# Autodesk Inventor assembly: Сборка_куб
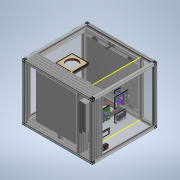
[picture p0: Inventor's stored thumbnail of the model, 180x180]
Saved by Autodesk Inventor 2020 (Build 240168000, 168)
## iProperties
Created: 2019-11-02
Part Number: Сборка_куб
Document SubType Name: Assembly
Designer: Михаил
Author: Михаил
## Documents named in this file (37)
- D:\MyWorks\GrowBox_v2\Box\3D_body\Сборка_куб.iam
- D:\MyWorks\GrowBox_v2\Box\3D_body\Профиль_аллюминиевый.ipt
- D:\MyWorks\GrowBox_v2\Box\3D_body\КубСоединительный2020.ipt
- D:\MyWorks\GrowBox_v2\Box\3D_body\Профиль_аллюминиевый460.ipt
- D:\MyWorks\GrowBox_v2\Box\3D_body\Профиль_аллюминиевый500.ipt
- D:\MyWorks\GrowBox_v2\Box\3D_body\Днище.ipt
- D:\MyWorks\GrowBox_v2\Box\3D_body\2004.ipt
- D:\MyWorks\GrowBox_v2\Box\3D_body\радиатор300х400.ipt
- D:\MyWorks\GrowBox_v2\Box\3D_body\ugolok40x40.ipt
- D:\MyWorks\GrowBox_v2\Box\3D_body\ugolok20x80.ipt
- D:\MyWorks\GrowBox_v2\Box\3D_body\petla.iam
- D:\MyWorks\GrowBox_v2\Box\3D_body\Uplotnitel-pazovyy400_-paz-6.ipt
- D:\MyWorks\GrowBox_v2\Box\3D_body\Uplotnitel-pazovyy380_-paz-6.ipt
- D:\MyWorks\GrowBox_v2\Box\3D_body\Uplotnitel-pazovyy500_-paz-6.ipt
- D:\MyWorks\GrowBox_v2\Box\3D_body\Дверка45.iam
- D:\MyWorks\GrowBox_v2\Box\3D_body\КрепежКулера.ipt
- D:\MyWorks\GrowBox_v2\Box\3D_body\NoctuaNF-A12x15.ipt
- D:\MyWorks\GrowBox_v2\Box\3D_body\КрепежРадиатора.ipt
- D:\MyWorks\GrowBox_v2\Box\3D_body\WaterContainer.ipt
- D:\MyWorks\GrowBox_v2\Box\3D_body\PowerSupply.ipt
- D:\MyWorks\GrowBox_v2\Box\3D_body\fitolamp_pcb.iam
- D:\MyWorks\GrowBox_v2\Box\3D_body\SensorsBoard.iam
- D:\MyWorks\GrowBox_v2\Box\3D_body\khadas-vim1-board.ipt
- D:\MyWorks\GrowBox_v2\Box\3D_body\Wall_Back_int.ipt
- D:\MyWorks\GrowBox_v2\Box\3D_body\DCDC_Holder.ipt
- D:\MyWorks\GrowBox_v2\Box\3D_body\FLC_Holder.ipt
- D:\MyWorks\GrowBox_v2\Box\3D_body\SensorsC_Holder.ipt
- D:\MyWorks\GrowBox_v2\Box\3D_body\SensorsBoard_3D\DA2_2.iam
- D:\MyWorks\GrowBox_v2\Box\3D_body\Wall_Input.ipt
- D:\MyWorks\GrowBox_v2\Box\3D_body\Wall_Output.ipt
- D:\MyWorks\GrowBox_v2\Box\3D_body\VIM1_Holder.ipt
- D:\MyWorks\GrowBox_v2\Box\3D_body\Wall_Front_door.ipt
- D:\MyWorks\GrowBox_v2\Box\3D_body\Разъем220.ipt
- D:\MyWorks\GrowBox_v2\Box\3D_body\Wall_Back_ext.ipt
- D:\MyWorks\GrowBox_v2\Box\3D_body\Wall_Top.ipt
- D:\MyWorks\GrowBox_v2\Box\3D_body\TempSensorHolder.ipt
- D:\MyWorks\GrowBox_v2\Box\3D_body\s-10-5_Holder.ipt
## Components (95 placed, 34 different names)
1. Профиль_алюминиевый:1 — Заподлицо:1, Заподлицо:2, Заподлицо:3, Совмещение:1, Заподлицо:4, Заподлицо:5, Совмещение:2, Заподлицо:6, Заподлицо:7
2. КубСоединительный2020:1 — Совмещение:1, Заподлицо:4, Заподлицо:5, Совмещение:6, Заподлицо:15, Совмещение:8, Заподлицо:18, Заподлицо:19, Заподлицо:20
3. КубСоединительный2020:2 — Совмещение:10, Заподлицо:23, Заподлицо:24, Совмещение:28, Заподлицо:50, Совмещение:29, Заподлицо:52, Заподлицо:53
4. КубСоединительный2020:3 — Совмещение:11, Заподлицо:25, Заподлицо:26, Заподлицо:51, Совмещение:30, Заподлицо:54, Заподлицо:55
5. КубСоединительный2020:4 — Совмещение:2, Заподлицо:6, Заподлицо:7, Совмещение:7, Заподлицо:16, Заподлицо:17, Совмещение:9, Заподлицо:21, Заподлицо:22
6. Профиль_алюминиевый:5 — Совмещение:7, Заподлицо:16, Заподлицо:17, Совмещение:13, Совмещение:15, Совмещение:16, Совмещение:34, Заподлицо:62, Заподлицо:63, Совмещение:53, Совмещение:91, Совмещение:104
7. Профиль_алюминиевый:6 — Совмещение:6, Заподлицо:15, Совмещение:31, Заподлицо:56, Заподлицо:57, Совмещение:56, Совмещение:71, Заподлицо:96, Совмещение:72, Заподлицо:97, Совмещение:85, Совмещение:96, Совмещение:105
8. Профиль_алюминиевый:7 — Совмещение:8, Заподлицо:18, Заподлицо:19, Заподлицо:20, Совмещение:10, Заподлицо:23, Заподлицо:24, Совмещение:20, Заподлицо:34, Заподлицо:35
9. Профиль_алюминиевый:8 — Совмещение:9, Заподлицо:21, Заподлицо:22, Совмещение:11, Заподлицо:25, Заподлицо:26, Совмещение:12, Заподлицо:27, Заподлицо:115
10. Профиль_алюминиевый:9 — Совмещение:12, Совмещение:13, Заподлицо:27, Совмещение:14, Заподлицо:28
11. Профиль_алюминиевый:10 — Совмещение:14, Совмещение:15, Заподлицо:28, Заподлицо:29, Совмещение:17, Совмещение:24, Заподлицо:43
12. Профиль_алюминиевый:11 — Совмещение:16, Заподлицо:29, Совмещение:17, Заподлицо:42, Заподлицо:86, Совмещение:54
13. Профиль_алюминиевый:12 — Заподлицо:32, Совмещение:20, Заподлицо:34, Заподлицо:35, Совмещение:114
14. Профиль_алюминиевый:13 — Заподлицо:32, Заподлицо:33
15. Профиль_алюминиевый:14 — Заподлицо:33, Совмещение:55, Заподлицо:87
16. Профиль_алюминиевый:15 — Заподлицо:36, Заподлицо:41, Совмещение:21, Совмещение:115, Заподлицо:116
17. Профиль_алюминиевый:16 — Заподлицо:36, Заподлицо:37, Заподлицо:40, Заподлицо:41, Совмещение:21, Совмещение:22, Совмещение:118
18. Профиль_алюминиевый:17 — Заподлицо:37, Заподлицо:38, Заподлицо:39, Заподлицо:40, Совмещение:22, Совмещение:23, Заподлицо:43
19. Профиль_алюминиевый:18 — Заподлицо:38, Заподлицо:39, Совмещение:23, Совмещение:24, Заподлицо:42, Совмещение:57, Заподлицо:88
20. Профиль_алюминиевый:19 — Заподлицо:50, Заподлицо:51
21. Профиль_алюминиевый:20 — Совмещение:28
22. Профиль_алюминиевый:21
23. Профиль_алюминиевый:22 — Совмещение:76, Заподлицо:99, Совмещение:144, Заподлицо:132
24. Профиль_алюминиевый:23 — Совмещение:30, Заподлицо:54, Заподлицо:55, Совмещение:33, Заподлицо:60, Заподлицо:61, Совмещение:79, Совмещение:89
25. Профиль_алюминиевый:24 — Совмещение:29, Заподлицо:52, Заподлицо:53, Совмещение:32, Заподлицо:58, Заподлицо:59, Совмещение:81, Совмещение:87
26. КубСоединительный2020:5 — Совмещение:34, Заподлицо:62, Заподлицо:63, Совмещение:35, Заподлицо:64, Заподлицо:65, Совмещение:92
27. КубСоединительный2020:6 — Совмещение:33, Заподлицо:60, Заподлицо:61, Совмещение:38, Заподлицо:70, Заподлицо:71, Совмещение:80, Совмещение:90, Совмещение:131
28. КубСоединительный2020:7 — Совмещение:32, Заподлицо:58, Заподлицо:59, Совмещение:37, Заподлицо:68, Заподлицо:69, Заподлицо:76, Совмещение:78, Совмещение:82, Совмещение:88
29. КубСоединительный2020:8 — Совмещение:31, Заподлицо:56, Заподлицо:57, Совмещение:36, Заподлицо:66, Заподлицо:67, Совмещение:86, Совмещение:129
30. Профиль_алюминиевый:25 — Совмещение:35, Заподлицо:64, Заподлицо:65, Совмещение:49, Заподлицо:84, Совмещение:97, Совмещение:109, Заподлицо:131
31. Профиль_алюминиевый:26 — Совмещение:36, Заподлицо:66, Заподлицо:67, Совмещение:44, Заподлицо:75, Заподлицо:76, Совмещение:45, Заподлицо:77, Совмещение:52, Совмещение:128, Заподлицо:130
32. Профиль_алюминиевый:27 — Совмещение:38, Заподлицо:70, Заподлицо:71, Совмещение:43, Заподлицо:74, Совмещение:50, Совмещение:103, Совмещение:117, Совмещение:130, Совмещение:143
33. Профиль_алюминиевый:28 — Совмещение:37, Заподлицо:68, Заподлицо:69, Совмещение:46, Совмещение:77, Заподлицо:129
34. Днище:1 — Совмещение:98, Совмещение:99, Совмещение:100
35. Профиль_алюминиевый:29 — Совмещение:45, Заподлицо:77, Совмещение:46, Заподлицо:78, Заподлицо:79, Совмещение:51, Заподлицо:85, Совмещение:84, Заподлицо:101
36. 2004:1 — Совмещение:43, Заподлицо:74, Заподлицо:79
37. 2004:2 — Совмещение:44, Заподлицо:75, Заподлицо:78
38. Профиль_алюминиевый:30 — Совмещение:47, Заподлицо:80, Заподлицо:81, Совмещение:49, Заподлицо:84, Совмещение:50
39. Профиль_алюминиевый:31 — Совмещение:47, Заподлицо:80, Заподлицо:81, Совмещение:108, Заподлицо:110
40. Профиль_алюминиевый:32 — Заподлицо:85, Совмещение:52, Совмещение:145, Заподлицо:133
41. Профиль_алюминиевый:33 — Совмещение:51
42. радиатор300х400:1 — Совмещение:108, Заподлицо:110, Совмещение:109, Совмещение:110, Заподлицо:111, Совмещение:111, Заподлицо:112, Совмещение:112, Заподлицо:113, Совмещение:113, Заподлицо:114
43. Профиль_алюминиевый:34 — Заподлицо:86, Совмещение:53, Совмещение:54, Совмещение:63, Заподлицо:89, Заподлицо:90, Совмещение:67, Совмещение:94, Заподлицо:103, Заподлицо:104, Заподлицо:127
44. Профиль_алюминиевый:35 — Совмещение:55, Заподлицо:87, Совмещение:56, Совмещение:58, Совмещение:64, Заподлицо:91, Совмещение:66, Заподлицо:92, Совмещение:93, Заподлицо:102, Совмещение:99, Совмещение:102, Заподлицо:105, Совмещение:116, Заподлицо:126
45. Профиль_алюминиевый:36 — Совмещение:57, Совмещение:58, Заподлицо:88, Совмещение:65, Совмещение:68, Заподлицо:93, Совмещение:69, Заподлицо:94, Совмещение:70, Заподлицо:95, Совмещение:83, Заподлицо:100, Совмещение:100, Заподлицо:125
46. ugolok40x40:1 — Совмещение:63, Заподлицо:89, Заподлицо:90
47. ugolok40x40:2 — Совмещение:67, Совмещение:68, Заподлицо:93
48. ugolok40x40:3 — Совмещение:65, Совмещение:66, Заподлицо:92
49. ugolok40x40:4 — Совмещение:64, Заподлицо:91, Совмещение:98
50. ugolok20x80:1 — Совмещение:69, Заподлицо:94
51. ugolok20x80:2 — Совмещение:70, Заподлицо:95
52. petla:1 [sub-assembly] — Совмещение:71, Заподлицо:96, Совмещение:95
53. petla:2 [sub-assembly] — Совмещение:72, Заподлицо:97
54. Uplotnitel-pazovyy400_-paz-6:1 — Совмещение:76, Заподлицо:99
55. Uplotnitel-pazovyy400_-paz-6:2 — Совмещение:77, Совмещение:78, Совмещение:142
56. Uplotnitel-pazovyy400_-paz-6:3 — Совмещение:79, Совмещение:80, Совмещение:141
57. Uplotnitel-pazovyy400_-paz-6:4 — Совмещение:81, Совмещение:82
58. Uplotnitel-pazovyy400_-paz-6:5 — Совмещение:83, Заподлицо:100
59. Uplotnitel-pazovyy400_-paz-6:6 — Совмещение:84, Заподлицо:101
60. Uplotnitel-pazovyy380_-paz-6:1 — Совмещение:87, Совмещение:88
61. Uplotnitel-pazovyy380_-paz-6:2 — Совмещение:85, Совмещение:86, Совмещение:133
62. Uplotnitel-pazovyy380_-paz-6:3 — Совмещение:89, Совмещение:90
63. Uplotnitel-pazovyy380_-paz-6:4 — Совмещение:91, Совмещение:92, Совмещение:135
64. Uplotnitel-pazovyy500_-paz-6:1 — Совмещение:93, Заподлицо:102, Совмещение:132
65. Uplotnitel-pazovyy500_-paz-6:2 — Совмещение:94, Заподлицо:103
66. Дверка45:1 [sub-assembly] — Совмещение:95, Совмещение:96, Совмещение:97, Совмещение:138, Совмещение:139, Заподлицо:128
67. КрепежКулера:1 — Совмещение:102, Заподлицо:105, Совмещение:105, Совмещение:107, Заподлицо:108, Заподлицо:109
68. КрепежКулера:2 — Заподлицо:104, Совмещение:103, Совмещение:104, Совмещение:106, Заподлицо:106, Заподлицо:107
69. NoctuaNF-A12x15:1 — Совмещение:106, Заподлицо:106, Заподлицо:107
70. NoctuaNF-A12x15:2 — Совмещение:107, Заподлицо:108, Заподлицо:109
71. КрепежРадиатора:1 — Совмещение:111, Заподлицо:112
72. КрепежРадиатора:2 — Совмещение:110, Заподлицо:111
73. КрепежРадиатора:3 — Совмещение:112, Заподлицо:113
74. КрепежРадиатора:4 — Совмещение:113, Заподлицо:114
75. WaterContainer:1 — Совмещение:114, Совмещение:115, Заподлицо:115
76. PowerSupply:1 — Совмещение:118, Заподлицо:116
77. fitolamp_pcb:1 [sub-assembly] — Совмещение:124, Заподлицо:117, Заподлицо:118
78. SensorsBoard:1 [sub-assembly] — Совмещение:126, Заподлицо:119, Заподлицо:120
79. khadas-vim1-board:1 — Совмещение:136, Заподлицо:123, Заподлицо:124
80. Wall_Back_int:1 — Совмещение:116, Совмещение:117, Совмещение:122, Совмещение:123, Совмещение:125, Совмещение:137, Совмещение:140, Заподлицо:125, Совмещение:146
81. DCDC_Holder:1 — Совмещение:122, Совмещение:127, Заподлицо:121, Заподлицо:122
82. FLC_Holder:1 — Совмещение:123, Совмещение:124, Заподлицо:117, Заподлицо:118
83. SensorsC_Holder:1 — Совмещение:125, Совмещение:126, Заподлицо:119, Заподлицо:120
84. DA2_2:1 [sub-assembly] — Совмещение:127, Заподлицо:121, Заподлицо:122
85. Uplotnitel-pazovyy500_-paz-6:3 — Совмещение:128, Совмещение:129
86. Uplotnitel-pazovyy500_-paz-6:4 — Совмещение:130, Совмещение:131, Совмещение:134
87. Wall_Input:1 — Совмещение:132, Совмещение:133, Совмещение:140, Заподлицо:126
88. Wall_Output:1 — Совмещение:134, Совмещение:135, Заподлицо:127
89. VIM1_Holder:1 — Совмещение:136, Заподлицо:123, Заподлицо:124, Совмещение:137
90. Wall_Front_door:1 — Совмещение:138, Совмещение:139, Заподлицо:128
91. Разъем220:1 — Совмещение:144, Заподлицо:132
92. Wall_Back_ext:1 — Заподлицо:129, Совмещение:141, Совмещение:142
93. Wall_Top:1 — Заподлицо:130, Совмещение:143, Заподлицо:131
94. TempSensorHolder:1 — Совмещение:145, Заподлицо:133
95. s-10-5_Holder:1 — Совмещение:146
## Relationships (251: Mate 128, Flush 123)
- Заподлицо:1 [Flush] (-6.75 mm): Профиль_алюминиевый:1
- Заподлицо:2 [Flush] (206.363 mm): Профиль_алюминиевый:1
- Заподлицо:3 [Flush] (17.615 mm): Профиль_алюминиевый:1
- Совмещение:1 [Mate]: Профиль_алюминиевый:1 ↔ КубСоединительный2020:1
- Заподлицо:4 [Flush]: Профиль_алюминиевый:1 ↔ КубСоединительный2020:1
- Заподлицо:5 [Flush]: Профиль_алюминиевый:1 ↔ КубСоединительный2020:1
- Совмещение:2 [Mate]: Профиль_алюминиевый:1 ↔ КубСоединительный2020:4
- Заподлицо:6 [Flush]: Профиль_алюминиевый:1 ↔ КубСоединительный2020:4
- Заподлицо:7 [Flush]: Профиль_алюминиевый:1 ↔ КубСоединительный2020:4
- Совмещение:6 [Mate]: КубСоединительный2020:1 ↔ Профиль_алюминиевый:6
- Заподлицо:15 [Flush]: КубСоединительный2020:1 ↔ Профиль_алюминиевый:6
- Совмещение:7 [Mate]: КубСоединительный2020:4 ↔ Профиль_алюминиевый:5
- Заподлицо:16 [Flush]: КубСоединительный2020:4 ↔ Профиль_алюминиевый:5
- Заподлицо:17 [Flush]: КубСоединительный2020:4 ↔ Профиль_алюминиевый:5
- Совмещение:8 [Mate]: КубСоединительный2020:1 ↔ Профиль_алюминиевый:7
- Заподлицо:18 [Flush]: КубСоединительный2020:1 ↔ Профиль_алюминиевый:7
- Заподлицо:19 [Flush]: КубСоединительный2020:1 ↔ Профиль_алюминиевый:7
- Заподлицо:20 [Flush]: КубСоединительный2020:1 ↔ Профиль_алюминиевый:7
- Совмещение:9 [Mate]: КубСоединительный2020:4 ↔ Профиль_алюминиевый:8
- Заподлицо:21 [Flush]: КубСоединительный2020:4 ↔ Профиль_алюминиевый:8
- Заподлицо:22 [Flush]: КубСоединительный2020:4 ↔ Профиль_алюминиевый:8
- Совмещение:10 [Mate]: КубСоединительный2020:2 ↔ Профиль_алюминиевый:7
- Заподлицо:23 [Flush]: КубСоединительный2020:2 ↔ Профиль_алюминиевый:7
- Заподлицо:24 [Flush]: КубСоединительный2020:2 ↔ Профиль_алюминиевый:7
- Совмещение:11 [Mate]: КубСоединительный2020:3 ↔ Профиль_алюминиевый:8
- Заподлицо:25 [Flush]: КубСоединительный2020:3 ↔ Профиль_алюминиевый:8
- Заподлицо:26 [Flush]: КубСоединительный2020:3 ↔ Профиль_алюминиевый:8
- Совмещение:12 [Mate]: Профиль_алюминиевый:8 ↔ Профиль_алюминиевый:9
- Совмещение:13 [Mate]: Профиль_алюминиевый:5 ↔ Профиль_алюминиевый:9
- Заподлицо:27 [Flush]: Профиль_алюминиевый:8 ↔ Профиль_алюминиевый:9
- Совмещение:14 [Mate]: Профиль_алюминиевый:9 ↔ Профиль_алюминиевый:10
- Совмещение:15 [Mate]: Профиль_алюминиевый:5 ↔ Профиль_алюминиевый:10
- Заподлицо:28 [Flush]: Профиль_алюминиевый:9 ↔ Профиль_алюминиевый:10
- Совмещение:16 [Mate]: Профиль_алюминиевый:5 ↔ Профиль_алюминиевый:11
- Заподлицо:29 [Flush]: Профиль_алюминиевый:10 ↔ Профиль_алюминиевый:11
- Совмещение:17 [Mate]: Профиль_алюминиевый:10 ↔ Профиль_алюминиевый:11
- [Mate]: Профиль_алюминиевый:12 ↔ Профиль_алюминиевый:13
- [Flush]: Профиль_алюминиевый:12 ↔ Профиль_алюминиевый:13
- [Flush]: Профиль_алюминиевый:13 ↔ Профиль_алюминиевый:14
- [Mate]: Профиль_алюминиевый:13 ↔ Профиль_алюминиевый:14
- Заподлицо:32 [Flush]: Профиль_алюминиевый:12 ↔ Профиль_алюминиевый:13
- Заподлицо:33 [Flush]: Профиль_алюминиевый:13 ↔ Профиль_алюминиевый:14
- Совмещение:20 [Mate]: Профиль_алюминиевый:7 ↔ Профиль_алюминиевый:12
- Заподлицо:34 [Flush]: Профиль_алюминиевый:7 ↔ Профиль_алюминиевый:12
- Заподлицо:35 [Flush]: Профиль_алюминиевый:7 ↔ Профиль_алюминиевый:12
- Заподлицо:36 [Flush]: Профиль_алюминиевый:15 ↔ Профиль_алюминиевый:16
- Заподлицо:37 [Flush]: Профиль_алюминиевый:16 ↔ Профиль_алюминиевый:17
- Заподлицо:38 [Flush]: Профиль_алюминиевый:17 ↔ Профиль_алюминиевый:18
- Заподлицо:39 [Flush]: Профиль_алюминиевый:17 ↔ Профиль_алюминиевый:18
- Заподлицо:40 [Flush]: Профиль_алюминиевый:16 ↔ Профиль_алюминиевый:17
- Заподлицо:41 [Flush]: Профиль_алюминиевый:15 ↔ Профиль_алюминиевый:16
- Совмещение:21 [Mate]: Профиль_алюминиевый:15 ↔ Профиль_алюминиевый:16
- Совмещение:22 [Mate]: Профиль_алюминиевый:16 ↔ Профиль_алюминиевый:17
- Совмещение:23 [Mate]: Профиль_алюминиевый:17 ↔ Профиль_алюминиевый:18
- Совмещение:24 [Mate]: Профиль_алюминиевый:10 ↔ Профиль_алюминиевый:18
- Заподлицо:42 [Flush]: Профиль_алюминиевый:11 ↔ Профиль_алюминиевый:18
- Заподлицо:43 [Flush] (80 mm): Профиль_алюминиевый:10 ↔ Профиль_алюминиевый:17
- [Flush]: Профиль_алюминиевый:19 ↔ Профиль_алюминиевый:20
- [Flush]: Профиль_алюминиевый:20 ↔ Профиль_алюминиевый:21
- [Flush]: Профиль_алюминиевый:21 ↔ Профиль_алюминиевый:22
- [Flush]: Профиль_алюминиевый:21 ↔ Профиль_алюминиевый:22
- [Flush]: Профиль_алюминиевый:20 ↔ Профиль_алюминиевый:21
- [Flush]: Профиль_алюминиевый:19 ↔ Профиль_алюминиевый:20
- [Mate]: Профиль_алюминиевый:19 ↔ Профиль_алюминиевый:20
- [Mate]: Профиль_алюминиевый:20 ↔ Профиль_алюминиевый:21
- [Mate]: Профиль_алюминиевый:21 ↔ Профиль_алюминиевый:22
- Совмещение:28 [Mate]: КубСоединительный2020:2 ↔ Профиль_алюминиевый:20
- Заподлицо:50 [Flush]: КубСоединительный2020:2 ↔ Профиль_алюминиевый:19
- Заподлицо:51 [Flush]: КубСоединительный2020:3 ↔ Профиль_алюминиевый:19
- Совмещение:29 [Mate]: КубСоединительный2020:2 ↔ Профиль_алюминиевый:24
- Заподлицо:52 [Flush]: КубСоединительный2020:2 ↔ Профиль_алюминиевый:24
- Заподлицо:53 [Flush]: КубСоединительный2020:2 ↔ Профиль_алюминиевый:24
- Совмещение:30 [Mate]: КубСоединительный2020:3 ↔ Профиль_алюминиевый:23
- Заподлицо:54 [Flush]: КубСоединительный2020:3 ↔ Профиль_алюминиевый:23
- Заподлицо:55 [Flush]: КубСоединительный2020:3 ↔ Профиль_алюминиевый:23
- Совмещение:31 [Mate]: Профиль_алюминиевый:6 ↔ КубСоединительный2020:8
- Заподлицо:56 [Flush]: Профиль_алюминиевый:6 ↔ КубСоединительный2020:8
- Заподлицо:57 [Flush]: Профиль_алюминиевый:6 ↔ КубСоединительный2020:8
- Совмещение:32 [Mate]: Профиль_алюминиевый:24 ↔ КубСоединительный2020:7
- Заподлицо:58 [Flush]: Профиль_алюминиевый:24 ↔ КубСоединительный2020:7
- Заподлицо:59 [Flush]: Профиль_алюминиевый:24 ↔ КубСоединительный2020:7
- Совмещение:33 [Mate]: Профиль_алюминиевый:23 ↔ КубСоединительный2020:6
- Заподлицо:60 [Flush]: Профиль_алюминиевый:23 ↔ КубСоединительный2020:6
- Заподлицо:61 [Flush]: Профиль_алюминиевый:23 ↔ КубСоединительный2020:6
- Совмещение:34 [Mate]: Профиль_алюминиевый:5 ↔ КубСоединительный2020:5
- Заподлицо:62 [Flush]: Профиль_алюминиевый:5 ↔ КубСоединительный2020:5
- Заподлицо:63 [Flush]: Профиль_алюминиевый:5 ↔ КубСоединительный2020:5
- Совмещение:35 [Mate]: КубСоединительный2020:5 ↔ Профиль_алюминиевый:25
- Заподлицо:64 [Flush]: КубСоединительный2020:5 ↔ Профиль_алюминиевый:25
- Заподлицо:65 [Flush]: КубСоединительный2020:5 ↔ Профиль_алюминиевый:25
- Совмещение:36 [Mate]: КубСоединительный2020:8 ↔ Профиль_алюминиевый:26
- Заподлицо:66 [Flush]: КубСоединительный2020:8 ↔ Профиль_алюминиевый:26
- Заподлицо:67 [Flush]: КубСоединительный2020:8 ↔ Профиль_алюминиевый:26
- Совмещение:37 [Mate]: КубСоединительный2020:7 ↔ Профиль_алюминиевый:28
- Заподлицо:68 [Flush]: КубСоединительный2020:7 ↔ Профиль_алюминиевый:28
- Заподлицо:69 [Flush]: КубСоединительный2020:7 ↔ Профиль_алюминиевый:28
- Совмещение:38 [Mate]: КубСоединительный2020:6 ↔ Профиль_алюминиевый:27
- Заподлицо:70 [Flush]: КубСоединительный2020:6 ↔ Профиль_алюминиевый:27
- Заподлицо:71 [Flush]: КубСоединительный2020:6 ↔ Профиль_алюминиевый:27
- Совмещение:43 [Mate]: Профиль_алюминиевый:27 ↔ 2004:1
- Заподлицо:74 [Flush] (-7 mm): Профиль_алюминиевый:27 ↔ 2004:1
- Совмещение:44 [Mate]: Профиль_алюминиевый:26 ↔ 2004:2
- Заподлицо:75 [Flush] (7 mm): Профиль_алюминиевый:26 ↔ 2004:2
- Заподлицо:76 [Flush]: КубСоединительный2020:7 ↔ Профиль_алюминиевый:26
- Совмещение:45 [Mate]: Профиль_алюминиевый:26 ↔ Профиль_алюминиевый:29
- Заподлицо:77 [Flush]: Профиль_алюминиевый:26 ↔ Профиль_алюминиевый:29
- Совмещение:46 [Mate] (80 mm): Профиль_алюминиевый:28 ↔ Профиль_алюминиевый:29
- Заподлицо:78 [Flush]: Профиль_алюминиевый:29 ↔ 2004:2
- Заподлицо:79 [Flush]: Профиль_алюминиевый:29 ↔ 2004:1
- Совмещение:47 [Mate]: Профиль_алюминиевый:30 ↔ Профиль_алюминиевый:31
- Заподлицо:80 [Flush]: Профиль_алюминиевый:30 ↔ Профиль_алюминиевый:31
- Заподлицо:81 [Flush]: Профиль_алюминиевый:30 ↔ Профиль_алюминиевый:31
- [Mate]: Профиль_алюминиевый:32 ↔ Профиль_алюминиевый:33
- [Flush]: Профиль_алюминиевый:32 ↔ Профиль_алюминиевый:33
- [Flush]: Профиль_алюминиевый:32 ↔ Профиль_алюминиевый:33
- Совмещение:49 [Mate]: Профиль_алюминиевый:25 ↔ Профиль_алюминиевый:30
- Заподлицо:84 [Flush]: Профиль_алюминиевый:25 ↔ Профиль_алюминиевый:30
- Совмещение:50 [Mate] (10 mm): Профиль_алюминиевый:27 ↔ Профиль_алюминиевый:30
- Совмещение:51 [Mate]: Профиль_алюминиевый:29 ↔ Профиль_алюминиевый:33
- Заподлицо:85 [Flush]: Профиль_алюминиевый:29 ↔ Профиль_алюминиевый:32
- Совмещение:52 [Mate] (10 mm): Профиль_алюминиевый:26 ↔ Профиль_алюминиевый:32
- Заподлицо:86 [Flush]: Профиль_алюминиевый:11 ↔ Профиль_алюминиевый:34
- Совмещение:53 [Mate]: Профиль_алюминиевый:5 ↔ Профиль_алюминиевый:34
- Совмещение:54 [Mate]: Профиль_алюминиевый:11 ↔ Профиль_алюминиевый:34
- Совмещение:55 [Mate]: Профиль_алюминиевый:14 ↔ Профиль_алюминиевый:35
- Заподлицо:87 [Flush]: Профиль_алюминиевый:14 ↔ Профиль_алюминиевый:35
- Совмещение:56 [Mate]: Профиль_алюминиевый:6 ↔ Профиль_алюминиевый:35
- Совмещение:57 [Mate]: Профиль_алюминиевый:18 ↔ Профиль_алюминиевый:36
- Совмещение:58 [Mate]: Профиль_алюминиевый:35 ↔ Профиль_алюминиевый:36
- Заподлицо:88 [Flush]: Профиль_алюминиевый:18 ↔ Профиль_алюминиевый:36
- Совмещение:63 [Mate]: Профиль_алюминиевый:34 ↔ ugolok40x40:1
- Заподлицо:89 [Flush]: Профиль_алюминиевый:34 ↔ ugolok40x40:1
- Заподлицо:90 [Flush]: Профиль_алюминиевый:34 ↔ ugolok40x40:1
- Совмещение:64 [Mate]: Профиль_алюминиевый:35 ↔ ugolok40x40:4
- Заподлицо:91 [Flush]: Профиль_алюминиевый:35 ↔ ugolok40x40:4
- Совмещение:65 [Mate]: Профиль_алюминиевый:36 ↔ ugolok40x40:3
- Совмещение:66 [Mate]: Профиль_алюминиевый:35 ↔ ugolok40x40:3
- Заподлицо:92 [Flush]: Профиль_алюминиевый:35 ↔ ugolok40x40:3
- Совмещение:67 [Mate]: Профиль_алюминиевый:34 ↔ ugolok40x40:2
- Совмещение:68 [Mate]: Профиль_алюминиевый:36 ↔ ugolok40x40:2
- Заподлицо:93 [Flush]: Профиль_алюминиевый:36 ↔ ugolok40x40:2
- Совмещение:69 [Mate]: Профиль_алюминиевый:36 ↔ ugolok20x80:1
- Заподлицо:94 [Flush]: Профиль_алюминиевый:36 ↔ ugolok20x80:1
- Совмещение:70 [Mate]: Профиль_алюминиевый:36 ↔ ugolok20x80:2
- Заподлицо:95 [Flush]: Профиль_алюминиевый:36 ↔ ugolok20x80:2
- Совмещение:71 [Mate]: Профиль_алюминиевый:6 ↔ petla:1
- Заподлицо:96 [Flush] (3 mm): Профиль_алюминиевый:6 ↔ petla:1
- Совмещение:72 [Mate]: Профиль_алюминиевый:6 ↔ petla:2
- Заподлицо:97 [Flush] (3 mm): Профиль_алюминиевый:6 ↔ petla:2
- Совмещение:76 [Mate]: Профиль_алюминиевый:22 ↔ Uplotnitel-pazovyy400_-paz-6:1
- Заподлицо:99 [Flush]: Профиль_алюминиевый:22 ↔ Uplotnitel-pazovyy400_-paz-6:1
- Совмещение:77 [Mate]: Профиль_алюминиевый:28 ↔ Uplotnitel-pazovyy400_-paz-6:2
- Совмещение:78 [Mate]: КубСоединительный2020:7 ↔ Uplotnitel-pazovyy400_-paz-6:2
- Совмещение:79 [Mate]: Профиль_алюминиевый:23 ↔ Uplotnitel-pazovyy400_-paz-6:3
- Совмещение:80 [Mate]: КубСоединительный2020:6 ↔ Uplotnitel-pazovyy400_-paz-6:3
- Совмещение:81 [Mate]: Профиль_алюминиевый:24 ↔ Uplotnitel-pazovyy400_-paz-6:4
- Совмещение:82 [Mate]: КубСоединительный2020:7 ↔ Uplotnitel-pazovyy400_-paz-6:4
- Совмещение:83 [Mate]: Профиль_алюминиевый:36 ↔ Uplotnitel-pazovyy400_-paz-6:5
- Заподлицо:100 [Flush]: Профиль_алюминиевый:36 ↔ Uplotnitel-pazovyy400_-paz-6:5
- Совмещение:84 [Mate]: Профиль_алюминиевый:29 ↔ Uplotnitel-pazovyy400_-paz-6:6
- Заподлицо:101 [Flush]: Профиль_алюминиевый:29 ↔ Uplotnitel-pazovyy400_-paz-6:6
- Совмещение:85 [Mate]: Профиль_алюминиевый:6 ↔ Uplotnitel-pazovyy380_-paz-6:2
- Совмещение:86 [Mate]: КубСоединительный2020:8 ↔ Uplotnitel-pazovyy380_-paz-6:2
- Совмещение:87 [Mate]: Профиль_алюминиевый:24 ↔ Uplotnitel-pazovyy380_-paz-6:1
- Совмещение:88 [Mate]: КубСоединительный2020:7 ↔ Uplotnitel-pazovyy380_-paz-6:1
- Совмещение:89 [Mate]: Профиль_алюминиевый:23 ↔ Uplotnitel-pazovyy380_-paz-6:3
- Совмещение:90 [Mate]: КубСоединительный2020:6 ↔ Uplotnitel-pazovyy380_-paz-6:3
- Совмещение:91 [Mate]: Профиль_алюминиевый:5 ↔ Uplotnitel-pazovyy380_-paz-6:4
- Совмещение:92 [Mate]: КубСоединительный2020:5 ↔ Uplotnitel-pazovyy380_-paz-6:4
- Совмещение:93 [Mate]: Профиль_алюминиевый:35 ↔ Uplotnitel-pazovyy500_-paz-6:1
- Заподлицо:102 [Flush]: Профиль_алюминиевый:35 ↔ Uplotnitel-pazovyy500_-paz-6:1
- Совмещение:94 [Mate]: Профиль_алюминиевый:34 ↔ Uplotnitel-pazovyy500_-paz-6:2
- Заподлицо:103 [Flush]: Профиль_алюминиевый:34 ↔ Uplotnitel-pazovyy500_-paz-6:2
- Совмещение:95 [Mate]: petla:1 ↔ Дверка45:1
- Совмещение:96 [Mate] (5 mm): Профиль_алюминиевый:6 ↔ Дверка45:1
- Совмещение:97 [Mate] (5 mm): Профиль_алюминиевый:25 ↔ Дверка45:1
- Совмещение:98 [Mate]: Днище:1 ↔ ugolok40x40:4
- Совмещение:99 [Mate]: Днище:1 ↔ Профиль_алюминиевый:35
- Совмещение:100 [Mate]: Днище:1 ↔ Профиль_алюминиевый:36
- Заподлицо:104 [Flush]: Профиль_алюминиевый:34 ↔ КрепежКулера:2
- Совмещение:102 [Mate]: Профиль_алюминиевый:35 ↔ КрепежКулера:1
- Заподлицо:105 [Flush]: Профиль_алюминиевый:35 ↔ КрепежКулера:1
- Совмещение:103 [Mate]: Профиль_алюминиевый:27 ↔ КрепежКулера:2
- Совмещение:104 [Mate] (140 mm): Профиль_алюминиевый:5 ↔ КрепежКулера:2
- Совмещение:105 [Mate] (134 mm): Профиль_алюминиевый:6 ↔ КрепежКулера:1
- Совмещение:106 [Mate]: КрепежКулера:2 ↔ NoctuaNF-A12x15:1
- Заподлицо:106 [Flush]: КрепежКулера:2 ↔ NoctuaNF-A12x15:1
- Заподлицо:107 [Flush]: КрепежКулера:2 ↔ NoctuaNF-A12x15:1
- Совмещение:107 [Mate]: КрепежКулера:1 ↔ NoctuaNF-A12x15:2
- Заподлицо:108 [Flush]: КрепежКулера:1 ↔ NoctuaNF-A12x15:2
- Заподлицо:109 [Flush]: КрепежКулера:1 ↔ NoctuaNF-A12x15:2
- Совмещение:108 [Mate]: Профиль_алюминиевый:31 ↔ радиатор300х400:1
- Заподлицо:110 [Flush]: Профиль_алюминиевый:31 ↔ радиатор300х400:1
- Совмещение:109 [Mate]: Профиль_алюминиевый:25 ↔ радиатор300х400:1
- Совмещение:110 [Mate]: радиатор300х400:1 ↔ КрепежРадиатора:2
- Заподлицо:111 [Flush]: радиатор300х400:1 ↔ КрепежРадиатора:2
- Совмещение:111 [Mate]: радиатор300х400:1 ↔ КрепежРадиатора:1
- Заподлицо:112 [Flush]: радиатор300х400:1 ↔ КрепежРадиатора:1
- Совмещение:112 [Mate]: радиатор300х400:1 ↔ КрепежРадиатора:3
- Заподлицо:113 [Flush]: радиатор300х400:1 ↔ КрепежРадиатора:3
- Совмещение:113 [Mate]: радиатор300х400:1 ↔ КрепежРадиатора:4
- Заподлицо:114 [Flush]: радиатор300х400:1 ↔ КрепежРадиатора:4
- Совмещение:114 [Mate]: Профиль_алюминиевый:12 ↔ WaterContainer:1
- Совмещение:115 [Mate]: Профиль_алюминиевый:15 ↔ WaterContainer:1
- Заподлицо:115 [Flush]: Профиль_алюминиевый:8 ↔ WaterContainer:1
- Совмещение:116 [Mate]: Профиль_алюминиевый:35 ↔ Wall_Back_int:1
- Совмещение:117 [Mate]: Профиль_алюминиевый:27 ↔ Wall_Back_int:1
- Совмещение:118 [Mate]: Профиль_алюминиевый:16 ↔ PowerSupply:1
- Заподлицо:116 [Flush]: Профиль_алюминиевый:15 ↔ PowerSupply:1
- Совмещение:122 [Mate]: Wall_Back_int:1 ↔ DCDC_Holder:1
- Совмещение:123 [Mate]: Wall_Back_int:1 ↔ FLC_Holder:1
- Совмещение:124 [Mate]: fitolamp_pcb:1 ↔ FLC_Holder:1
- Заподлицо:117 [Flush]: fitolamp_pcb:1 ↔ FLC_Holder:1
- Заподлицо:118 [Flush]: fitolamp_pcb:1 ↔ FLC_Holder:1
- Совмещение:125 [Mate]: Wall_Back_int:1 ↔ SensorsC_Holder:1
- Совмещение:126 [Mate]: SensorsBoard:1 ↔ SensorsC_Holder:1
- Заподлицо:119 [Flush]: SensorsBoard:1 ↔ SensorsC_Holder:1
- Заподлицо:120 [Flush]: SensorsBoard:1 ↔ SensorsC_Holder:1
- Совмещение:127 [Mate]: DCDC_Holder:1 ↔ DA2_2:1
- Заподлицо:121 [Flush]: DCDC_Holder:1 ↔ DA2_2:1
- Заподлицо:122 [Flush]: DCDC_Holder:1 ↔ DA2_2:1
- Совмещение:128 [Mate]: Профиль_алюминиевый:26 ↔ Uplotnitel-pazovyy500_-paz-6:3
- Совмещение:129 [Mate]: КубСоединительный2020:8 ↔ Uplotnitel-pazovyy500_-paz-6:3
- Совмещение:130 [Mate]: Профиль_алюминиевый:27 ↔ Uplotnitel-pazovyy500_-paz-6:4
- Совмещение:131 [Mate]: КубСоединительный2020:6 ↔ Uplotnitel-pazovyy500_-paz-6:4
- Совмещение:132 [Mate] (1.2 mm): Uplotnitel-pazovyy500_-paz-6:1 ↔ Wall_Input:1
- Совмещение:133 [Mate] (1.2 mm): Uplotnitel-pazovyy380_-paz-6:2 ↔ Wall_Input:1
- Совмещение:134 [Mate] (1.2 mm): Uplotnitel-pazovyy500_-paz-6:4 ↔ Wall_Output:1
- Совмещение:135 [Mate] (1.2 mm): Uplotnitel-pazovyy380_-paz-6:4 ↔ Wall_Output:1
- Совмещение:136 [Mate]: khadas-vim1-board:1 ↔ VIM1_Holder:1
- Заподлицо:123 [Flush]: khadas-vim1-board:1 ↔ VIM1_Holder:1
- Заподлицо:124 [Flush]: khadas-vim1-board:1 ↔ VIM1_Holder:1
- Совмещение:137 [Mate]: Wall_Back_int:1 ↔ VIM1_Holder:1
- Совмещение:138 [Mate]: Дверка45:1 ↔ Wall_Front_door:1
- Совмещение:139 [Mate]: Дверка45:1 ↔ Wall_Front_door:1
- Совмещение:140 [Mate]: Wall_Back_int:1 ↔ Wall_Input:1
- Заподлицо:125 [Flush] (-8 mm): Профиль_алюминиевый:36 ↔ Wall_Back_int:1
- Заподлицо:126 [Flush] (-8 mm): Профиль_алюминиевый:35 ↔ Wall_Input:1
- Заподлицо:127 [Flush] (-8 mm): Профиль_алюминиевый:34 ↔ Wall_Output:1
- Заподлицо:128 [Flush] (-8 mm): Дверка45:1 ↔ Wall_Front_door:1
- Заподлицо:129 [Flush] (-8 mm): Профиль_алюминиевый:28 ↔ Wall_Back_ext:1
- Совмещение:141 [Mate] (1.2 mm): Uplotnitel-pazovyy400_-paz-6:3 ↔ Wall_Back_ext:1
- Совмещение:142 [Mate] (1.2 mm): Uplotnitel-pazovyy400_-paz-6:2 ↔ Wall_Back_ext:1
- Заподлицо:130 [Flush]: Профиль_алюминиевый:26 ↔ Wall_Top:1
- Совмещение:143 [Mate]: Профиль_алюминиевый:27 ↔ Wall_Top:1
- Заподлицо:131 [Flush]: Профиль_алюминиевый:25 ↔ Wall_Top:1
- Совмещение:144 [Mate]: Профиль_алюминиевый:22 ↔ Разъем220:1
- Заподлицо:132 [Flush]: Профиль_алюминиевый:22 ↔ Разъем220:1
- Совмещение:145 [Mate]: Профиль_алюминиевый:32 ↔ TempSensorHolder:1
- Заподлицо:133 [Flush]: Профиль_алюминиевый:32 ↔ TempSensorHolder:1
- Совмещение:146 [Mate]: Wall_Back_int:1 ↔ s-10-5_Holder:1
## Named parameters: d51_d45 = 0 mm, d52_d47 = 0 mm, d53_d49 = 0 mm, d54_d50 = 0 mm, d72_d60 = 0 mm, d73_d61 = 0 mm, d74_d62 = 0 mm, d75_d63 = 0 mm, d76_d64 = 0 mm, d77_d65 = 0 mm, d78_d66 = 0 mm, d79_d67 = 0 mm, d80_d68 = 0 mm, d139_d138 = 0 mm, d140_d136 = 0 mm, d141_d137 = 0 mm
